# Autodesk Inventor assembly: gearbox_assembly
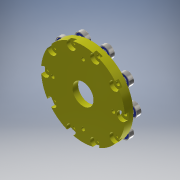
[picture p0: Inventor's stored thumbnail of the model, 180x180]
Saved by Autodesk Inventor 2019 (Build 230136000, 136)
## iProperties
Created: 2019-12-22
Part Number: gearbox_assembly
Material: Типовые
Document SubType Name: Assembly
Designer: Петров Иван
Author: Петров Иван
## Documents named in this file (3)
- E:\IVAN\Ivan_desktop\Kvantorium\ROBOTS\Arm_manip\hardware\gearbox_assembly.iam
- E:\IVAN\Ivan_desktop\Kvantorium\ROBOTS\Arm_manip\hardware\gearbox_down.ipt
- E:\IVAN\Ivan_desktop\Kvantorium\ROBOTS\Arm_manip\hardware\Standart_things\Подшипник 624Z.ipt
## Components (11 placed, 2 different names)
1. gearbox_down:1 — Совмещение:1, Совмещение:2, Совмещение:3, Совмещение:4, Совмещение:5, Совмещение:6, Совмещение:7, Совмещение:8, Совмещение:9, Совмещение:10, Совмещение:11, Совмещение:12, Совмещение:13, Совмещение:14, Совмещение:15, Совмещение:16, Совмещение:17, Совмещение:18, Совмещение:19, Совмещение:20
2. Подшипник 624Z:1 — Совмещение:1, Совмещение:2
3. Подшипник 624Z:2 — Совмещение:3, Совмещение:4
4. Подшипник 624Z:3 — Совмещение:5, Совмещение:6
5. Подшипник 624Z:4 — Совмещение:7, Совмещение:8
6. Подшипник 624Z:5 — Совмещение:9, Совмещение:10
7. Подшипник 624Z:6 — Совмещение:11, Совмещение:12
8. Подшипник 624Z:7 — Совмещение:13, Совмещение:14
9. Подшипник 624Z:8 — Совмещение:15, Совмещение:16
10. Подшипник 624Z:9 — Совмещение:17, Совмещение:18
11. Подшипник 624Z:10 — Совмещение:19, Совмещение:20
## Relationships (20: Mate 20)
- Совмещение:1 [Mate]: gearbox_down:1 ↔ Подшипник 624Z:1
- Совмещение:2 [Mate] (1 mm): gearbox_down:1 ↔ Подшипник 624Z:1
- Совмещение:3 [Mate] (1 mm): gearbox_down:1 ↔ Подшипник 624Z:2
- Совмещение:4 [Mate]: gearbox_down:1 ↔ Подшипник 624Z:2
- Совмещение:5 [Mate] (1 mm): gearbox_down:1 ↔ Подшипник 624Z:3
- Совмещение:6 [Mate]: gearbox_down:1 ↔ Подшипник 624Z:3
- Совмещение:7 [Mate] (1 mm): gearbox_down:1 ↔ Подшипник 624Z:4
- Совмещение:8 [Mate]: gearbox_down:1 ↔ Подшипник 624Z:4
- Совмещение:9 [Mate] (1 mm): gearbox_down:1 ↔ Подшипник 624Z:5
- Совмещение:10 [Mate]: gearbox_down:1 ↔ Подшипник 624Z:5
- Совмещение:11 [Mate] (1 mm): gearbox_down:1 ↔ Подшипник 624Z:6
- Совмещение:12 [Mate]: gearbox_down:1 ↔ Подшипник 624Z:6
- Совмещение:13 [Mate] (1 mm): gearbox_down:1 ↔ Подшипник 624Z:7
- Совмещение:14 [Mate]: gearbox_down:1 ↔ Подшипник 624Z:7
- Совмещение:15 [Mate] (1 mm): gearbox_down:1 ↔ Подшипник 624Z:8
- Совмещение:16 [Mate]: gearbox_down:1 ↔ Подшипник 624Z:8
- Совмещение:17 [Mate] (1 mm): gearbox_down:1 ↔ Подшипник 624Z:9
- Совмещение:18 [Mate]: gearbox_down:1 ↔ Подшипник 624Z:9
- Совмещение:19 [Mate] (1 mm): gearbox_down:1 ↔ Подшипник 624Z:10
- Совмещение:20 [Mate]: gearbox_down:1 ↔ Подшипник 624Z:10
